# Autodesk Inventor assembly: Body 2.0
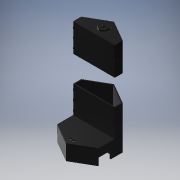
[picture p0: Inventor's stored thumbnail of the model, 180x180]
Saved by Autodesk Inventor 2017 (Build 210142000, 142)
## iProperties
Created: 2019-05-22
Part Number: Body 2.0
Document SubType Name: Assembly
Designer: Dell
Mass: 15253.7 g
Surface Area: 41598.8 cm^2
Volume: 19269.8 cm^3
Density: 0.791585 g/cm^3
Author: Dell
## Documents named in this file (19)
- C:\Users\Dell\Documents\GitHub\tr2\Body 2.0\Body 2.0.iam
- C:\Users\Dell\Documents\GitHub\tr2\Body 2.0\BA01.ipt
- C:\Users\Dell\Documents\GitHub\tr2\Body 2.0\BA02.ipt
- C:\Users\Dell\Documents\GitHub\tr2\Body 2.0\BA03.ipt
- C:\Users\Dell\Documents\GitHub\tr2\Body 2.0\BA04.ipt
- C:\Users\Dell\Documents\GitHub\tr2\Body 2.0\BA05.ipt
- C:\Users\Dell\Documents\GitHub\tr2\Body 2.0\BA06.ipt
- C:\Users\Dell\Documents\GitHub\tr2\Body 2.0\BA07.ipt
- C:\Users\Dell\Documents\GitHub\tr2\Body 2.0\BA08.ipt
- C:\Users\Dell\Documents\GitHub\tr2\Body 2.0\ST01.ipt
- C:\Users\Dell\Documents\GitHub\tr2\Actuator 1.3\Actuator 1.3.iam
- C:\Users\Dell\Documents\GitHub\tr2\Body 2.0\AE01.ipt
- C:\Users\Dell\Documents\GitHub\tr2\Body 2.0\BA09.ipt
- C:\Users\Dell\Documents\GitHub\tr2\Body 2.0\BA10.ipt
- C:\Users\Dell\Documents\GitHub\tr2\Body 2.0\BA11.ipt
- C:\Users\Dell\Documents\GitHub\tr2\Body 2.0\BA12.ipt
- C:\Users\Dell\Documents\GitHub\tr2\Body 2.0\BA13.ipt
- C:\Users\Dell\Documents\GitHub\tr2\Body 2.0\BA14.ipt
- C:\Users\Dell\Documents\GitHub\tr2\Body 2.0\BA15.ipt
## Components (22 placed, 18 different names)
1. BA01:1 — Mate:1, Flush:1, Flush:2, Mate:2, Flush:3, Flush:4, Mate:4, Flush:5, Mate:10, Flush:11, Mate:52
2. BA02:1 — Mate:1, Flush:1, Flush:2, Mate:3, Mate:9, Mate:13, Mate:14, Mate:36, Mate:37, Mate:38, Flush:13
3. BA03:1 — Mate:2, Mate:3, Flush:3, Mate:5, Mate:15, Mate:31
4. BA04:1 — Flush:4, Mate:4, Mate:5, Mate:7, Mate:32, Mate:39, Mate:40, Mate:41, Flush:19, Flush:26
5. BA05:1 — Flush:5, Mate:7, Mate:33, Mate:34, Mate:35, Flush:17, Mate:52
6. BA06:1 — Mate:9, Mate:10, Mate:12, Flush:11, Flush:14
7. BA07:1 — Mate:12, Mate:13, Mate:26, Mate:27, Flush:9, Flush:10, Mate:28, Mate:29, Mate:30, Flush:26
8. BA08:1 — Mate:14, Mate:15, Mate:21, Mate:23, Mate:24, Mate:25, Mate:31
9. ST01:1 — Mate:32, Mate:39, Mate:40, Mate:41
10. ST01:2 — Mate:33, Mate:34, Mate:35
11. ST01:3 — Mate:21, Mate:36, Mate:37, Mate:38
12. Actuator 1.3:1 [sub-assembly] — Mate:23, Mate:24, Mate:25
13. AE01:1 — Mate:27, Flush:9, Mate:29
14. AE01:2 — Mate:26, Flush:10, Mate:28, Mate:30
15. BA09:1 — Flush:13, Flush:15, Flush:16, Mate:42, Flush:21, Mate:46, Flush:22, Mate:51
16. BA10:1 — Flush:14, Flush:15, Flush:16, Mate:42, Flush:18, Mate:43, Flush:23, Mate:47, Flush:25
17. BA11:1 — Flush:17, Flush:18, Mate:43, Flush:20, Mate:44
18. BA12:1 — Flush:19, Flush:20, Mate:44
19. BA13:1 — Flush:21, Mate:46, Flush:22, Flush:24, Mate:48, Mate:50
20. BA14:1 — Flush:23, Mate:47, Mate:49
21. BA14:2 — Flush:24, Mate:48, Mate:49
22. BA15:1 — Mate:50, Flush:25, Mate:51
## Relationships (64: Mate 42, Flush 22)
- Mate:1: BA01:1 ↔ BA02:1
- Flush:1: BA01:1 ↔ BA02:1
- Flush:2: BA01:1 ↔ BA02:1
- Mate:2: BA01:1 ↔ BA03:1
- Mate:3: BA02:1 ↔ BA03:1
- Flush:3: BA01:1 ↔ BA03:1
- Flush:4: BA01:1 ↔ BA04:1
- Mate:4: BA01:1 ↔ BA04:1
- Mate:5: BA03:1 ↔ BA04:1
- Flush:5: BA01:1 ↔ BA05:1
- Mate:7: BA04:1 ↔ BA05:1
- Mate:9: BA02:1 ↔ BA06:1
- Mate:10: BA01:1 ↔ BA06:1
- Mate:12 (1.27 mm): BA06:1 ↔ BA07:1
- Mate:13 (1.27 mm): BA02:1 ↔ BA07:1
- Mate:14 (1.27 mm): BA02:1 ↔ BA08:1
- Mate:15 (1.27 mm): BA03:1 ↔ BA08:1
- Mate:21: BA08:1 ↔ ST01:3
- Mate:23: BA08:1 ↔ Actuator 1.3:1
- Mate:24: BA08:1 ↔ Actuator 1.3:1
- Mate:25: BA08:1 ↔ Actuator 1.3:1
- Mate:26: BA07:1 ↔ AE01:2
- Mate:27: BA07:1 ↔ AE01:1
- Flush:9: BA07:1 ↔ AE01:1
- Flush:10: BA07:1 ↔ AE01:2
- Mate:28: BA07:1 ↔ AE01:2
- Mate:29: BA07:1 ↔ AE01:1
- Mate:30: BA07:1 ↔ AE01:2
- Flush:11: BA01:1 ↔ BA06:1
- Mate:31 (1.27 mm): BA03:1 ↔ BA08:1
- Mate:32: BA04:1 ↔ ST01:1
- Mate:33: BA05:1 ↔ ST01:2
- Mate:34: BA05:1 ↔ ST01:2
- Mate:35: BA05:1 ↔ ST01:2
- Mate:36: BA02:1 ↔ ST01:3
- Mate:37: BA02:1 ↔ ST01:3
- Mate:38: BA02:1 ↔ ST01:3
- Mate:39: BA04:1 ↔ ST01:1
- Mate:40: BA04:1 ↔ ST01:1
- Mate:41: BA04:1 ↔ ST01:1
- Flush:13: BA02:1 ↔ BA09:1
- Flush:14: BA06:1 ↔ BA10:1
- Flush:15: BA09:1 ↔ BA10:1
- Flush:16: BA09:1 ↔ BA10:1
- Mate:42: BA09:1 ↔ BA10:1
- Flush:17: BA05:1 ↔ BA11:1
- Flush:18: BA10:1 ↔ BA11:1
- Mate:43: BA10:1 ↔ BA11:1
- Flush:19: BA04:1 ↔ BA12:1
- Flush:20: BA11:1 ↔ BA12:1
- Mate:44: BA11:1 ↔ BA12:1
- Flush:21: BA09:1 ↔ BA13:1
- Mate:46: BA09:1 ↔ BA13:1
- Flush:22: BA09:1 ↔ BA13:1
- Flush:23: BA10:1 ↔ BA14:1
- Mate:47: BA10:1 ↔ BA14:1
- Flush:24: BA13:1 ↔ BA14:2
- Mate:48: BA13:1 ↔ BA14:2
- Mate:49: BA14:1 ↔ BA14:2
- Mate:50: BA13:1 ↔ BA15:1
- Flush:25: BA10:1 ↔ BA15:1
- Mate:51: BA09:1 ↔ BA15:1
- Mate:52: BA01:1 ↔ BA05:1
- Flush:26: BA04:1 ↔ BA07:1
## Named parameters: Panel_Thickness = 6.35 mm, Fit_Tolerance = 1.27 mm, Tool_Dia = 6.35 mm, iTrigger0 = 1
